# Autodesk Inventor assembly: robot arm
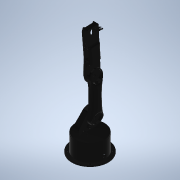
[picture p0: Inventor's stored thumbnail of the model, 180x180]
Saved by Autodesk Inventor 2022 (Build 260153000, 153)
## iProperties
Created: 2021-06-19
Part Number: robot arm
Document SubType Name: Assembly
Designer: fanam
Author: fanam
## Documents named in this file (6)
- C:\Users\fanam\Documents\robot arm.iam
- C:\Users\fanam\Desktop\Imported Components\Waist\Waist.ipt
- C:\Users\fanam\Desktop\Imported Components\Gripper\Gripper.ipt
- C:\Users\fanam\Desktop\Imported Components\Base\Base.ipt
- C:\Users\fanam\Desktop\Imported Components\Arm 02\Arm 02.ipt
- C:\Users\fanam\Desktop\Imported Components\Arm 01\Arm 01.ipt
## Components (5 placed, 5 different names)
1. Waist:1 — Rotational:1, Rotational:2
2. Gripper:1 — Rotational:4
3. Base:1 — Rotational:1
4. Arm 02:1 — Rotational:3, Rotational:4
5. Arm 01:1 — Rotational:2, Rotational:3
## Relationships (4: RevoluteJoint 4)
- Rotational:1 [RevoluteJoint]: Waist:1 ↔ Base:1
- Rotational:2 [RevoluteJoint]: Waist:1 ↔ Arm 01:1
- Rotational:3 [RevoluteJoint]: Arm 02:1 ↔ Arm 01:1
- Rotational:4 [RevoluteJoint]: Gripper:1 ↔ Arm 02:1
